# Autodesk Inventor assembly: Faulhaber 3272G012C R
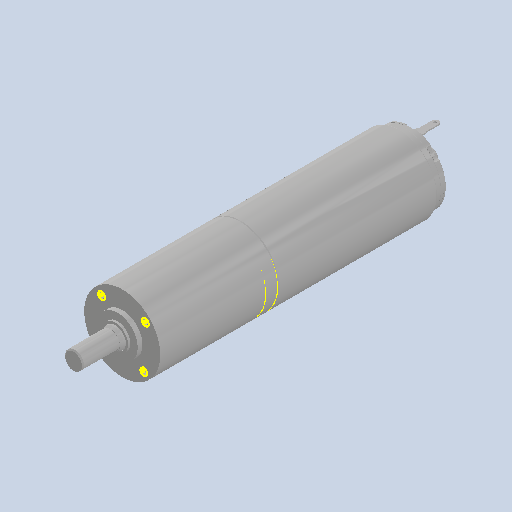
[picture p0: Inventor's stored thumbnail of the model, 512x512]
Saved by Autodesk Inventor 2022 (Build 260153000, 153)
## iProperties
Created: 2023-01-02
Part Number: Faulhaber 3272G012C R
Document SubType Name: Assembly
Designer: komputer
Author: komputer
## Documents named in this file (4)
- D:\konarm 2 przegub\Faulhaber 3272G012C R.iam
- D:\Konarm_1_przegub_final\32-3_flange_c.ipt
- D:\Konarm_1_przegub_final\32-3_3stage.ipt
- D:\Konarm_1_przegub_final\3272G_CR.ipt
## Components (3 placed, 3 different names)
1. 32-3_flange_c:1 — Mate:1, Mate:2
2. 32-3_3stage:1 — Mate:3, Mate:4
3. 3272G_CR:1 — Mate:1, Mate:2, Mate:3, Mate:4
## Relationships (4: Mate 4)
- Mate:1: 32-3_flange_c:1 ↔ 3272G_CR:1
- Mate:2: 32-3_flange_c:1 ↔ 3272G_CR:1
- Mate:3: 32-3_3stage:1 ↔ 3272G_CR:1
- Mate:4: 32-3_3stage:1 ↔ 3272G_CR:1
